# Autodesk Inventor assembly: A-31-08P-1300
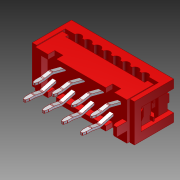
[picture p0: Inventor's stored thumbnail of the model, 180x180]
Saved by Autodesk Inventor 2014 (Build 180170000, 170)
## iProperties
Company: TraceParts S.A.
Created: 2013-08-30
Part Number: A-31-08P-1300
Checked By: TraceParts S.A.
Catalog Web Link: www.traceparts.com
Description: Micro-Miniature Steckverbinder, 8 polig, Raster 1,27mm, IDC
Vendor: ASSMANN WSW components
Document SubType Name: Assembly
Designer: TraceParts
TraceParts.PartNumber: 10-16062010-082809
TraceParts.ClassPath: ASSMANN:/ROOT/10-16062010-082809
TraceParts.InstanceId: 10-16062010-082809C5X08N8DVADMC5NSP0VJH1X5K
REFERENCE: A-31-08P-1300
TRACEPARTS: TRACEPARTS
SUPPLIER: ASSMANN WSW components
DESIGN: Micro-Miniature Steckverbinder, 8 polig, Raster 1,27mm, IDC
TraceParts.PartStatus: Published
TraceParts.PartVersion: 1.1.4
Title: Micro-Miniature Steckverbinder, 8 polig, Raster 1,27mm, IDC
Author: TraceParts
## Documents named in this file (3)
- C:\Users\Felix\Desktop\Beep\Hardware\3D-CAD\parts\electronic\BEEP\components\micro-miniature_steckverbinder_a-31-08p-1300.iam
- C:\Users\Felix\Desktop\Beep\Hardware\3D-CAD\parts\electronic\BEEP\components\micro-miniature_steckverbinder_a-31-08p-1300_02.ipt
- C:\Users\Felix\Desktop\Beep\Hardware\3D-CAD\parts\electronic\BEEP\components\micro-miniature_steckverbinder_a-31-08p-1300_01.ipt
## Components (2 placed, 2 different names)
1. micro-miniature_steckverbinder_a-31-08p-1300_02:1 — Passend:1, Passend:2, Fluchtend:1
2. micro-miniature_steckverbinder_a-31-08p-1300_01:1 — Passend:1, Passend:2, Fluchtend:1
## Relationships (3: Mate 2, Flush 1)
- Passend:1 [Mate]: micro-miniature_steckverbinder_a-31-08p-1300_02:1 ↔ micro-miniature_steckverbinder_a-31-08p-1300_01:1
- Passend:2 [Mate] (0.1 mm): micro-miniature_steckverbinder_a-31-08p-1300_02:1 ↔ micro-miniature_steckverbinder_a-31-08p-1300_01:1
- Fluchtend:1 [Flush]: micro-miniature_steckverbinder_a-31-08p-1300_02:1 ↔ micro-miniature_steckverbinder_a-31-08p-1300_01:1
